# Autodesk Inventor assembly: COMPLETE ASSEMBLY
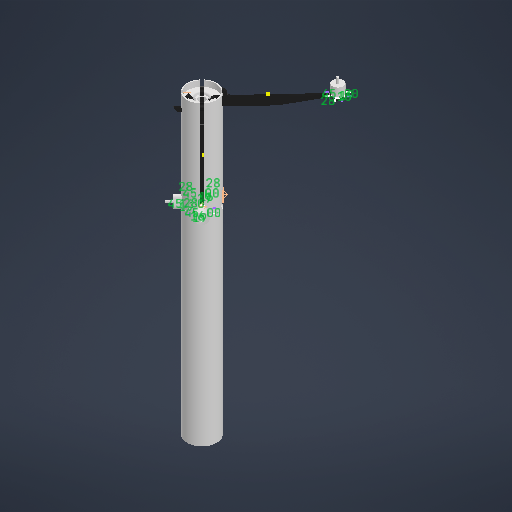
[picture p0: Inventor's stored thumbnail of the model, 512x512]
Saved by Autodesk Inventor 2025 (Build 290162010, 162A)
## iProperties
Created: 2025-07-06
Part Number: COMPLETE ASSEMBLY
Document SubType Name: Assembly
Designer: Jebediah Kerman
Author: Jebediah Kerman
## Documents named in this file (4)
- F:\Desktop\Projects\RTLS_VIC\CAD\COMPLETE ASSEMBLY.iam
- F:\Desktop\Projects\RTLS_VIC\CAD\BOOM ASSEMBLY.iam
- F:\Desktop\Projects\RTLS_VIC\CAD\CENTER RING.ipt
- F:\Desktop\Projects\RTLS_VIC\CAD\ROCKET BODY.ipt
## Components (6 placed, 3 different names)
1. BOOM ASSEMBLY:1 [sub-assembly] — Rotational:1
2. BOOM ASSEMBLY:2 [sub-assembly] — Rotational:2
3. BOOM ASSEMBLY:3 [sub-assembly] — Rotational:3
4. BOOM ASSEMBLY:4 [sub-assembly] — Rotational:4
5. CENTER RING:1 — Rotational:1, Rotational:2, Rotational:3, Rotational:4, Mate:1, Flush:1
6. ROCKET BODY:1 — Mate:1, Flush:1
## Relationships (6: RevoluteJoint 4, Mate 1, Flush 1)
- Rotational:1 [RevoluteJoint] (-2 mm): BOOM ASSEMBLY:1 ↔ CENTER RING:1
- Rotational:2 [RevoluteJoint] (-2 mm): BOOM ASSEMBLY:2 ↔ CENTER RING:1
- Rotational:3 [RevoluteJoint] (-2 mm): BOOM ASSEMBLY:3 ↔ CENTER RING:1
- Rotational:4 [RevoluteJoint] (-2 mm): BOOM ASSEMBLY:4 ↔ CENTER RING:1
- Mate:1: CENTER RING:1 ↔ ROCKET BODY:1
- Flush:1 (14 mm): CENTER RING:1 ↔ ROCKET BODY:1
